# Autodesk Inventor assembly: FunkschalterV01.1
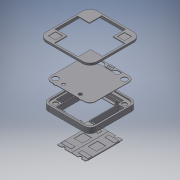
[picture p0: Inventor's stored thumbnail of the model, 180x180]
Saved by Autodesk Inventor 2016 SP2 (Build 200236200, 236)
## iProperties
Created: 2018-06-26
Part Number: FunkschalterV01.1
Material: Generisch
Document SubType Name: Assembly
Designer: Nils
Author: Nils
## Documents named in this file (6)
- C:\Users\Nils\Documents\Inventor\Funkschalter\V01.2\FunkschalterV01.2.iam
- C:\Users\Nils\Documents\Inventor\Funkschalter\V01.2\Bauteil1.ipt
- C:\Users\Nils\Documents\Inventor\Funkschalter\V01.2\Boden.ipt
- C:\Users\Nils\Documents\Inventor\Funkschalter\V01.2\Button.ipt
- C:\Users\Nils\Documents\Inventor\Funkschalter\V01.2\Wandhalterung.ipt
- C:\Users\Nils\Documents\Inventor\Funkschalter\V01.2\Button_MIR.ipt
## Components (5 placed, 5 different names)
1. Bauteil1:1 — Passend:3, Passend:5, Passend:6
2. Boden:1 — Passend:3
3. Button:1 — Fluchtend:1, Fluchtend:2, Fluchtend:3, Passend:6
4. Wandhalterung:1 — Passend:5
5. Button_MIR:1 — Passend:4, Fluchtend:2, Fluchtend:3
## Relationships (7: Mate 4, Flush 3)
- Passend:3 [Mate] (17.399 mm): Bauteil1:1 ↔ Boden:1
- Fluchtend:1 [Flush] (0.1 mm): Button:1
- Passend:4 [Mate] (0.1 mm): Button_MIR:1
- Passend:5 [Mate] (129.967 mm): Bauteil1:1 ↔ Wandhalterung:1
- Fluchtend:2 [Flush]: Button:1 ↔ Button_MIR:1
- Fluchtend:3 [Flush]: Button:1 ↔ Button_MIR:1
- Passend:6 [Mate] (-28.251 mm): Bauteil1:1 ↔ Button:1
